# Autodesk Inventor assembly: POM_T5_28
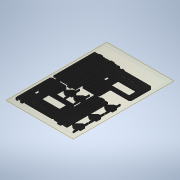
[picture p0: Inventor's stored thumbnail of the model, 180x180]
Saved by Autodesk Inventor 2020 (Build 240168000, 168)
## iProperties
Created: 2021-08-27
Part Number: POM_T5_28
Document SubType Name: Assembly
Designer: Masato
Author: Masato
## Documents named in this file (7)
- C:\Inventor\SUSTAINA-OP\Cam\POM_T5_28.iam
- C:\Inventor\SUSTAINA-OP\Cam\DisposableBoard.ipt
- C:\Inventor\SUSTAINA-OP\UpperBody\Cockpit\Cockpit_side_frame.ipt
- C:\Inventor\SUSTAINA-OP\UpperBody\Head\Camera_side_frame.ipt
- C:\Inventor\SUSTAINA-OP\UpperBody\Cockpit\Cockpit_battery_bottom_frame.ipt
- C:\Inventor\SUSTAINA-OP\UpperBody\Cockpit\Cockpit_battery_front_frame.ipt
- C:\Inventor\SUSTAINA-OP\UpperBody\Cockpit\Cockpit_side_frame_MIR.ipt
## Components (11 placed, 6 different names)
1. DisposableBoard:1 — メイト:2, メイト:1, フラッシュ:1, フラッシュ:2, メイト:4, フラッシュ:3, フラッシュ:4, メイト:13, メイト:14, メイト:16, メイト:19, メイト:21
2. Cockpit_side_frame:1 — メイト:4, フラッシュ:3, フラッシュ:4, フラッシュ:5, メイト:17, フラッシュ:6, メイト:18, フラッシュ:7, メイト:23
3. Cockpit_battery_bottom_frame:1 — メイト:16, フラッシュ:5, メイト:17, 正接:1, メイト:22, メイト:24
4. Cockpit_side_frame_MIR:1 — メイト:19, メイト:20, メイト:24
5. Cockpit_battery_front_frame:1 — メイト:14, メイト:18, フラッシュ:7
6. Cockpit_battery_front_frame:2 — メイト:20
7. Camera_side_frame:2 — メイト:13, フラッシュ:6, 正接:1
8. Camera_side_frame:3
9. Camera_side_frame:4
10. Camera_side_frame:6 — メイト:21, メイト:22, メイト:23
11. Camera_side_frame:7
## Component patterns: (2 elements, first: Cockpit_battery_front_frame:1), (3 elements, first: Camera_side_frame:2), (2 elements, first: Camera_side_frame:6)
## Relationships (22: Mate 14, Flush 7, Tangent 1)
- メイト:2 [Mate]: DisposableBoard:1
- メイト:1 [Mate]: DisposableBoard:1
- フラッシュ:1 [Flush]: DisposableBoard:1
- フラッシュ:2 [Flush]: DisposableBoard:1
- メイト:4 [Mate]: DisposableBoard:1 ↔ Cockpit_side_frame:1
- フラッシュ:3 [Flush] (2 mm): DisposableBoard:1 ↔ Cockpit_side_frame:1
- フラッシュ:4 [Flush] (2 mm): DisposableBoard:1 ↔ Cockpit_side_frame:1
- メイト:13 [Mate]: DisposableBoard:1 ↔ Camera_side_frame:2
- メイト:14 [Mate]: DisposableBoard:1 ↔ Cockpit_battery_front_frame:1
- メイト:16 [Mate]: DisposableBoard:1 ↔ Cockpit_battery_bottom_frame:1
- フラッシュ:5 [Flush]: Cockpit_side_frame:1 ↔ Cockpit_battery_bottom_frame:1
- メイト:17 [Mate] (2.1 mm): Cockpit_side_frame:1 ↔ Cockpit_battery_bottom_frame:1
- フラッシュ:6 [Flush]: Cockpit_side_frame:1 ↔ Camera_side_frame:2
- 正接:1 [Tangent] (2.1 mm): Cockpit_battery_bottom_frame:1 ↔ Camera_side_frame:2
- メイト:18 [Mate] (2.5 mm): Cockpit_side_frame:1 ↔ Cockpit_battery_front_frame:1
- フラッシュ:7 [Flush]: Cockpit_side_frame:1 ↔ Cockpit_battery_front_frame:1
- メイト:19 [Mate]: DisposableBoard:1 ↔ Cockpit_side_frame_MIR:1
- メイト:20 [Mate] (2.5 mm): Cockpit_side_frame_MIR:1 ↔ Cockpit_battery_front_frame:2
- メイト:21 [Mate]: DisposableBoard:1 ↔ Camera_side_frame:6
- メイト:22 [Mate] (2.5 mm): Cockpit_battery_bottom_frame:1 ↔ Camera_side_frame:6
- メイト:23 [Mate] (2.5 mm): Cockpit_side_frame:1 ↔ Camera_side_frame:6
- メイト:24 [Mate] (2.5 mm): Cockpit_battery_bottom_frame:1 ↔ Cockpit_side_frame_MIR:1
